# Autodesk Inventor assembly: 4483T461_HIGH-STRENGTH BALL JOINT ROD END
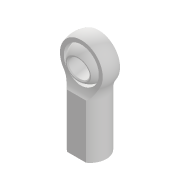
[picture p0: Inventor's stored thumbnail of the model, 180x180]
Saved by Autodesk Inventor 2021 (Build 250183000, 183)
## iProperties
Created: 2021-05-08
Part Number: 4483T461_HIGH-STRENGTH BALL JOINT ROD END
Document SubType Name: Assembly
Designer: Santiago Suárez
Author: Santiago Suárez
## Documents named in this file (3)
- C:\Users\Santiago Suárez\Documents\GitHub\Dis.-Mecatronico-E6\inventor proyecto\4483T461_HIGH-STRENGTH BALL JOINT ROD END.iam
- C:\Users\Santiago Suárez\Documents\GitHub\Dis.-Mecatronico-E6\inventor proyecto\Solid2.ipt
- C:\Users\Santiago Suárez\Documents\GitHub\Dis.-Mecatronico-E6\inventor proyecto\Solid1.ipt
## Components (2 placed, 2 different names)
1. Solid2:1 — Ball:1
2. Solid1:1 — Ball:1
## Relationships (1: BallJoint 1)
- Ball:1: Solid2:1 ↔ Solid1:1
